# Autodesk Inventor assembly: motor unit
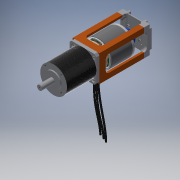
[picture p0: Inventor's stored thumbnail of the model, 180x180]
Saved by Autodesk Inventor 2018 (Build 220112000, 112)
## iProperties
Created: 2019-12-10
Part Number: motor unit
Document SubType Name: Assembly
Designer: Bunny320
Author: Bunny320
## Documents named in this file (11)
- C:\Users\Bunny320\Desktop\sechs\4-CAD\motor unit.iam
- C:\Users\Bunny320\Desktop\sechs\4-CAD\901-4250 house.ipt
- C:\Users\Bunny320\Desktop\sechs\4-CAD\911-42-reducer-long.ipt
- C:\Users\Bunny320\Desktop\sechs\4-CAD\standardParts\turnigy sk3 4250 350kv\BLDC Motor Turnigy Aerodrive SK3 350KV Outrunner.iam
- C:\Users\Bunny320\Desktop\sechs\4-CAD\902-4250 magnet hold.ipt
- C:\Users\Bunny320\Desktop\sechs\4-CAD\magnet-6x2.5.ipt
- C:\Users\Bunny320\Desktop\sechs\4-CAD\AS5047.ipt
- C:\Users\Bunny320\Desktop\sechs\4-CAD\903-4250 back.ipt
- C:\Users\Bunny320\Documents\Inventor\Content Center Files\R2018\en-US\DIN 7991(2)\DIN 7991 - M3x12.ipt
- C:\Users\Bunny320\Documents\Inventor\Content Center Files\R2018\en-US\ISO 4762(1)\DIN EN ISO 4762 - M2 x 6.ipt
- C:\Users\Bunny320\Documents\Inventor\Content Center Files\R2018\en-US\DIN EN ISO 4032\DIN EN ISO 4032 - M2.ipt
## Components (19 placed, 10 different names)
1. 901-4250 house:1 — Flush:1, Flush:2, Flush:3, Mate:1, Mate:2, Mate:3, Mate:4, Flush:4, Flush:5, Flush:6, Mate:10
2. 911-42-reducer-long:1 — Mate:3, Mate:4, Flush:4, Mate:14, Mate:15, Mate:16, Mate:17
3. BLDC Motor Turnigy Aerodrive SK3 350KV Outrunner:1 [sub-assembly] — Mate:1, Mate:2, Mate:5, Mate:6
4. 902-4250 magnet hold:1 — Mate:5, Mate:6, Mate:7, Mate:8
5. magnet-6x2.5:1 — Mate:7, Mate:8
6. AS5047:1 — Mate:11, Mate:12, Mate:13, Mate:19, Mate:21, Mate:23, Mate:25
7. 903-4250 back:1 — Flush:5, Flush:6, Mate:10, Mate:11, Mate:12, Mate:13, Mate:18, Mate:20, Mate:22, Mate:24, Insert:1, Insert:2, Insert:3, Insert:4
8. DIN 7991 M3x12:1 — Mate:14
9. DIN 7991 M3x12:2 — Mate:15
10. DIN 7991 M3x12:3 — Mate:16
11. DIN 7991 M3x12:4 — Mate:17
12. DIN EN ISO 4762 M2 x 6:1 — Mate:18, Mate:19
13. DIN EN ISO 4762 M2 x 6:2 — Mate:20, Mate:21
14. DIN EN ISO 4762 M2 x 6:3 — Mate:22, Mate:23
15. DIN EN ISO 4762 M2 x 6:4 — Mate:24, Mate:25
16. DIN EN ISO 4032 M2:1 — Insert:1
17. DIN EN ISO 4032 M2:2 — Insert:2
18. DIN EN ISO 4032 M2:3 — Insert:3
19. DIN EN ISO 4032 M2:4 — Insert:4
## Relationships (34: Mate 24, Flush 6, Insert 4)
- Flush:1: 901-4250 house:1
- Flush:2: 901-4250 house:1
- Flush:3: 901-4250 house:1
- Mate:1: 901-4250 house:1 ↔ BLDC Motor Turnigy Aerodrive SK3 350KV Outrunner:1
- Mate:2: 901-4250 house:1 ↔ BLDC Motor Turnigy Aerodrive SK3 350KV Outrunner:1
- Mate:3: 901-4250 house:1 ↔ 911-42-reducer-long:1
- Mate:4: 901-4250 house:1 ↔ 911-42-reducer-long:1
- Flush:4: 901-4250 house:1 ↔ 911-42-reducer-long:1
- Mate:5: BLDC Motor Turnigy Aerodrive SK3 350KV Outrunner:1 ↔ 902-4250 magnet hold:1
- Mate:6: BLDC Motor Turnigy Aerodrive SK3 350KV Outrunner:1 ↔ 902-4250 magnet hold:1
- Mate:7: 902-4250 magnet hold:1 ↔ magnet-6x2.5:1
- Mate:8: 902-4250 magnet hold:1 ↔ magnet-6x2.5:1
- Flush:5: 901-4250 house:1 ↔ 903-4250 back:1
- Flush:6: 901-4250 house:1 ↔ 903-4250 back:1
- Mate:10: 901-4250 house:1 ↔ 903-4250 back:1
- Mate:11: AS5047:1 ↔ 903-4250 back:1
- Mate:12: AS5047:1 ↔ 903-4250 back:1
- Mate:13: AS5047:1 ↔ 903-4250 back:1
- Mate:14: 911-42-reducer-long:1 ↔ DIN 7991 M3x12:1
- Mate:15: 911-42-reducer-long:1 ↔ DIN 7991 M3x12:2
- Mate:16: 911-42-reducer-long:1 ↔ DIN 7991 M3x12:3
- Mate:17: 911-42-reducer-long:1 ↔ DIN 7991 M3x12:4
- Mate:18: 903-4250 back:1 ↔ DIN EN ISO 4762 M2 x 6:1
- Mate:19: AS5047:1 ↔ DIN EN ISO 4762 M2 x 6:1
- Mate:20: 903-4250 back:1 ↔ DIN EN ISO 4762 M2 x 6:2
- Mate:21: AS5047:1 ↔ DIN EN ISO 4762 M2 x 6:2
- Mate:22: 903-4250 back:1 ↔ DIN EN ISO 4762 M2 x 6:3
- Mate:23: AS5047:1 ↔ DIN EN ISO 4762 M2 x 6:3
- Mate:24: 903-4250 back:1 ↔ DIN EN ISO 4762 M2 x 6:4
- Mate:25: AS5047:1 ↔ DIN EN ISO 4762 M2 x 6:4
- Insert:1: 903-4250 back:1 ↔ DIN EN ISO 4032 M2:1
- Insert:2: 903-4250 back:1 ↔ DIN EN ISO 4032 M2:2
- Insert:3: 903-4250 back:1 ↔ DIN EN ISO 4032 M2:3
- Insert:4: 903-4250 back:1 ↔ DIN EN ISO 4032 M2:4
